# Autodesk Inventor assembly: RBMk2Assembly
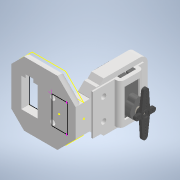
[picture p0: Inventor's stored thumbnail of the model, 180x180]
Saved by Autodesk Inventor 2020 (Build 240168000, 168)
## iProperties
Created: 2020-03-20
Part Number: RBMk2Assembly
Document SubType Name: Assembly
Designer: varun
Author: varun
## iProperties of the stored document MG90servo_shaft.ipt
Created: 2016-03-21
Part Number: MG90servo_shaft
Material: Generic
Document SubType Name: Modeling
Designer: varun
Density: 1 g/cm^3
Appearance: Default
Author: varun
Sending System: SolidWorks 2015
Last Author: Vitto
Last Saved: 2016-03-21
## iProperties of the stored document MG90servo_gear.ipt
Created: 2016-03-21
Part Number: MG90servo_gear
Material: Generic
Document SubType Name: Modeling
Designer: varun
Density: 1 g/cm^3
Appearance: Default
Author: varun
Sending System: SolidWorks 2015
Last Author: Vitto
Last Saved: 2016-03-21
## iProperties of the stored document MG90servo_assembly.iam
Created: 2016-03-21
Part Number: MG90servo_assembly
Document SubType Name: Assembly
Designer: varun
Author: varun
Sending System: SolidWorks 2015
Last Author: Vitto
Last Saved: 2016-03-21
## iProperties of the stored document MG90servo_body.ipt
Created: 2016-03-21
Part Number: MG90servo_body
Material: Generic
Document SubType Name: Modeling
Designer: varun
Density: 1 g/cm^3
Appearance: Default
Author: varun
Sending System: SolidWorks 2015
Last Author: Vitto
Last Saved: 2016-03-21
## Documents named in this file (11)
- **C:\Users\varun\Desktop\ServoArm\RBMk2Assembly.iam*LocalDocs*xAaaaaldaAaaaaaaaAaaaqrggKd*MG90servo_shaft.ipt
- **C:\Users\varun\Desktop\ServoArm\RBMk2Assembly.iam*LocalDocs*xAaaaaidaAaaaaaaaAaaaaljaJh*MG90servo_gear.ipt
- **C:\Users\varun\Desktop\ServoArm\RBMk2Assembly.iam*LocalDocs*xAaaaaedaAaaaaaaaAaaaqgv5Yg*MG90servo_assembly.iam
- **C:\Users\varun\Desktop\ServoArm\RBMk2Assembly.iam*LocalDocs*xAaaaqkbaAaaaaaaaAaaaqgphCf*MG90servo_body.ipt
- C:\Users\varun\Desktop\ServoArm\RBMk2Assembly.iam
- C:\Users\varun\Desktop\ServoArm\Rotator Base mk2.ipt
- C:\Users\varun\Desktop\ServoArm\Servo Holder Cap.ipt
- C:\Users\varun\Desktop\ServoArm\MG90servo_assembly.SLDASM
- C:\Users\varun\Desktop\ServoArm\MG90servo_body.SLDPRT
- C:\Users\varun\Desktop\ServoArm\MG90servo_gear.SLDPRT
- C:\Users\varun\Desktop\ServoArm\MG90servo_shaft.SLDPRT
## Components (3 placed, 3 different names)
1. MG90servo_assembly:1 [sub-assembly] — Mate:1, Mate:2, Mate:3, Mate:5, Mate:6
2. Rotator Base mk2:1 — Mate:1, Mate:2, Mate:3, Mate:4
3. Servo Holder Cap:1 — Mate:4, Mate:5, Mate:6
## Relationships (6: Mate 6)
- Mate:1: MG90servo_assembly:1 ↔ Rotator Base mk2:1
- Mate:2: MG90servo_assembly:1 ↔ Rotator Base mk2:1
- Mate:3: MG90servo_assembly:1 ↔ Rotator Base mk2:1
- Mate:4: Rotator Base mk2:1 ↔ Servo Holder Cap:1
- Mate:5: MG90servo_assembly:1 ↔ Servo Holder Cap:1
- Mate:6: MG90servo_assembly:1 ↔ Servo Holder Cap:1
